# Autodesk Inventor assembly: x_motor
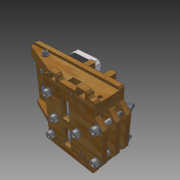
[picture p0: Inventor's stored thumbnail of the model, 180x180]
Saved by Autodesk Inventor 2014 (Build 180170000, 170)
## iProperties
Created: 2014-04-03
Part Number: x_motor
Document SubType Name: Assembly
Designer: buben
Author: buben
## Documents named in this file (23)
- C:\Users\buben\Documents\GitHub\bacon\inventor files\assemblies\x_motor.iam
- C:\Users\buben\Documents\GitHub\bacon\inventor files\printer parts\x_motor_back.ipt
- C:\Users\buben\Documents\GitHub\bacon\inventor files\printer parts\x_motor_cable_mount.ipt
- C:\Users\buben\Documents\GitHub\bacon\inventor files\printer parts\x_motor_cable_mount_brace.ipt
- C:\Users\buben\Documents\GitHub\bacon\inventor files\printer parts\x_motor_smooth_rod_spacer.ipt
- C:\Users\buben\Documents\GitHub\bacon\inventor files\printer parts\x_motor_wall_upper.ipt
- C:\Users\buben\Documents\GitHub\bacon\inventor files\printer parts\x_motor_wall_lower.ipt
- C:\Users\buben\Documents\GitHub\bacon\inventor files\printer parts\x_motor_upper_nut_stop.ipt
- C:\Users\buben\Documents\GitHub\bacon\inventor files\printer parts\motor_spacer.ipt
- C:\Users\buben\Documents\GitHub\bacon\inventor files\utils\washer_m4.ipt
- C:\Users\buben\Documents\Inventor\Content Center Files\R2014\en-US\ISO 4762(2)\ISO 4762 - M4 x 20ISO.ipt
- C:\Users\buben\Documents\Inventor\Content Center Files\R2014\en-US\ISO 7040\ISO 7040 - M4.ipt
- C:\Users\buben\Documents\GitHub\bacon\inventor files\printer parts\x_motor_middle.ipt
- C:\Users\buben\Documents\Inventor\Content Center Files\R2014\en-US\CSN EN 24032\ISO 4032 - M5CSN EN.ipt
- C:\Users\buben\Documents\GitHub\bacon\inventor files\3rd party components\linear_bearing_8\Imported Components\LU8MM\LU8MM.iam
- C:\Users\buben\Documents\GitHub\bacon\inventor files\printer parts\x_motor_top.ipt
- C:\Users\buben\Documents\GitHub\bacon\inventor files\printer parts\x_motor_lower_nut_stop.ipt
- C:\Users\buben\Documents\GitHub\bacon\inventor files\utils\washer_m5.ipt
- C:\Users\buben\Documents\Inventor\Content Center Files\R2014\en-US\ISO 7040\ISO 7040 - M5.ipt
- C:\Users\buben\Documents\Inventor\Content Center Files\R2014\en-US\ISO 4762(2)\ISO 4762 - M5 x 50ISO.ipt
- C:\Users\buben\Documents\GitHub\bacon\inventor files\utils\washer_m3.ipt
- C:\Users\buben\Documents\Inventor\Content Center Files\R2014\en-US\ISO 4762(2)\ISO 4762 - M3 x 20ISO.ipt
- C:\Users\buben\Documents\GitHub\bacon\inventor files\3rd party components\nema_17_stepper\Imported Components\NEMA 17 with T5 Pulley\NEMA 17 with T5 Pulley.iam
## Components (77 placed, 22 different names)
1. x_motor_back:1 — Mate:1, Mate:2, Mate:3, Mate:4, Mate:5, Mate:6, Mate:8, Mate:10, Mate:11, Mate:12, Mate:13, Mate:14, Mate:15, Mate:16, Mate:17, Mate:18, Mate:19, Mate:20, Mate:21, Mate:22, Mate:23, Mate:24, Mate:25, Tangent:1, Tangent:2, Mate:26, Mate:27, Mate:40, Mate:41, Mate:74, Mate:75, Mate:76, Mate:77, Mate:78, Mate:79, Mate:106, Mate:109, Mate:112, Mate:115
2. x_motor_cable_mount:1 — Mate:4, Mate:5, Mate:6, Mate:7, Mate:9, Mate:30, Mate:38, Mate:39
3. x_motor_cable_mount_brace:1 — Mate:7, Mate:8, Mate:9, Mate:42, Mate:44
4. x_motor_smooth_rod_spacer:1 — Mate:10, Mate:13, Mate:14
5. x_motor_smooth_rod_spacer:2 — Mate:11, Mate:12, Mate:15
6. x_motor_wall_upper:1 — Mate:16, Mate:17, Mate:18, Mate:32, Mate:50, Mate:54, Mate:55
7. x_motor_wall_lower:1 — Mate:19, Mate:20, Mate:21, Mate:51, Mate:52, Mate:56, Mate:57, Flush:1, Mate:63, Mate:64, Mate:67, Flush:2, Mate:125, Mate:126, Mate:127, Mate:128
8. x_motor_upper_nut_stop:1 — Mate:22, Mate:23, Mate:24, Mate:28, Mate:29, Mate:53
9. motor_spacer:1 — Mate:25, Tangent:1, Tangent:2, Mate:116, Mate:117, Mate:118, Mate:119, Mate:120, Mate:121, Mate:122
10. CSN 02 1702 B B 4,3:1 — Mate:28, Mate:29, Insert:1
11. CSN 02 1702 B B 4,3:2 — Mate:26, Mate:27, Insert:2
12. CSN 02 1702 B B 4,3:3 — Mate:32, Mate:33, Mate:34
13. CSN 02 1702 B B 4,3:4 — Mate:30, Mate:31, Mate:36
14. ISO 4762 M4 x 20:1 — Insert:2, Mate:31, Mate:37
15. ISO 4762 M4 x 20:2 — Insert:1, Mate:33, Mate:35
16. DIN EN ISO 7040 M4:1 — Mate:36, Mate:37
17. DIN EN ISO 7040 M4:2 — Mate:34, Mate:35
18. CSN 02 1702 B B 4,3:5 — Mate:44, Mate:45, Mate:48
19. CSN 02 1702 B B 4,3:6 — Mate:42, Mate:43, Mate:46
20. CSN 02 1702 B B 4,3:7 — Mate:38, Mate:39, Insert:4
21. CSN 02 1702 B B 4,3:8 — Mate:40, Mate:41, Insert:3
22. ISO 4762 M4 x 20:3 — Insert:4, Mate:43, Mate:47
23. ISO 4762 M4 x 20:4 — Insert:3, Mate:45, Mate:49
24. DIN EN ISO 7040 M4:3 — Mate:48, Mate:49
25. DIN EN ISO 7040 M4:4 — Mate:46, Mate:47
26. x_motor_middle:1 — Mate:50, Mate:51, Mate:52, Mate:58, Mate:59, Mate:60, Mate:62, Mate:66
27. CSN EN 24032 M5:1 — Mate:53, Mate:54, Mate:55
28. CSN EN 24032 M5:2 — Mate:56, Mate:57, Flush:1
29. LU8MM:1 [sub-assembly] — Mate:58, Mate:59, Mate:60, Mate:61
30. LU8MM:2 [sub-assembly] — Mate:61, Mate:62, Mate:65
31. x_motor_top:1 — Mate:63, Mate:64, Mate:65, Mate:68, Mate:69, Mate:70, Mate:71, Mate:72, Mate:73, Mate:80, Mate:81, Mate:82, Mate:83, Mate:84, Mate:85
32. x_motor_lower_nut_stop:1 — Mate:66, Mate:67, Flush:2, Mate:123, Mate:124
33. CSN 02 1702 B B 5,3:1 — Mate:72, Mate:83, Insert:7
34. CSN 02 1702 B B 5,3:2 — Mate:76, Mate:87, Mate:94
35. CSN 02 1702 B B 5,3:3 — Mate:77, Mate:91, Mate:102
36. CSN 02 1702 B B 5,3:4 — Mate:79, Mate:89, Mate:100
37. CSN 02 1702 B B 5,3:5 — Mate:78, Mate:90, Mate:98
38. CSN 02 1702 B B 5,3:6 — Mate:75, Mate:88, Mate:96
39. CSN 02 1702 B B 5,3:7 — Mate:74, Mate:86, Mate:92
40. CSN 02 1702 B B 5,3:8 — Mate:73, Mate:84, Insert:5
41. CSN 02 1702 B B 5,3:9 — Mate:71, Mate:85, Insert:9
42. CSN 02 1702 B B 5,3:10 — Mate:70, Mate:82, Insert:10
43. CSN 02 1702 B B 5,3:11 — Mate:69, Mate:81, Insert:8
44. CSN 02 1702 B B 5,3:12 — Mate:68, Mate:80, Insert:6
45. ISO 4762 M5 x 50:1 — Insert:10, Mate:86, Mate:93
46. ISO 4762 M5 x 50:4 — Insert:9, Mate:89, Mate:101
47. ISO 4762 M5 x 50:3 — Insert:8, Mate:88, Mate:97
48. ISO 4762 M5 x 50:5 — Insert:7, Mate:90, Mate:99
49. ISO 4762 M5 x 50:2 — Insert:6, Mate:87, Mate:95
50. ISO 4762 M5 x 50:6 — Insert:5, Mate:91, Mate:103
51. DIN EN ISO 7040 M5:1 — Mate:100, Mate:101
52. DIN EN ISO 7040 M5:2 — Mate:98, Mate:99
53. DIN EN ISO 7040 M5:3 — Mate:96, Mate:97
54. DIN EN ISO 7040 M5:4 — Mate:92, Mate:93
55. DIN EN ISO 7040 M5:5 — Mate:102, Mate:103
56. DIN EN ISO 7040 M5:6 — Mate:94, Mate:95
57. CSN 02 1702 B B 3,2:1 — Mate:110, Mate:111, Insert:13
58. CSN 02 1702 B B 3,2:2 — Mate:107, Mate:108, Insert:12
59. CSN 02 1702 B B 3,2:3 — Mate:110, Mate:111, Mate:112
60. CSN 02 1702 B B 3,2:4 — Mate:113, Mate:114, Insert:14
61. CSN 02 1702 B B 3,2:5 — Mate:113, Mate:114, Mate:115
62. CSN 02 1702 B B 3,2:6 — Mate:107, Mate:108, Mate:109
63. CSN 02 1702 B B 3,2:7 — Mate:104, Mate:105
64. CSN 02 1702 B B 3,2:8 — Mate:104, Mate:105, Mate:106, Insert:11
65. ISO 4762 M3 x 20:1 — Insert:14, Mate:122
66. ISO 4762 M3 x 20:2 — Insert:13, Mate:119
67. ISO 4762 M3 x 20:3 — Insert:12, Mate:120
68. ISO 4762 M3 x 20:4 — Insert:11, Mate:121
69. NEMA 17 with T5 Pulley:1 [sub-assembly] — Mate:116, Mate:117, Mate:118
70. CSN 02 1702 B B 4,3:9 — Mate:126, Mate:127, Insert:16
71. CSN 02 1702 B B 4,3:10 — Mate:125, Mate:128, Insert:15
72. CSN 02 1702 B B 4,3:11 — Mate:124, Mate:130, Mate:133
73. CSN 02 1702 B B 4,3:12 — Mate:123, Mate:129, Mate:131
74. ISO 4762 M4 x 20:5 — Insert:16, Mate:130, Mate:134
75. ISO 4762 M4 x 20:6 — Insert:15, Mate:129, Mate:132
76. DIN EN ISO 7040 M4:5 — Mate:133, Mate:134
77. DIN EN ISO 7040 M4:6 — Mate:131, Mate:132
## Relationships (154: Mate 134, Insert 16, Tangent 2, Flush 2)
- Mate:1: x_motor_back:1
- Mate:2: x_motor_back:1
- Mate:3: x_motor_back:1
- Mate:4: x_motor_back:1 ↔ x_motor_cable_mount:1
- Mate:5: x_motor_back:1 ↔ x_motor_cable_mount:1
- Mate:6: x_motor_back:1 ↔ x_motor_cable_mount:1
- Mate:7: x_motor_cable_mount:1 ↔ x_motor_cable_mount_brace:1
- Mate:8: x_motor_back:1 ↔ x_motor_cable_mount_brace:1
- Mate:9: x_motor_cable_mount:1 ↔ x_motor_cable_mount_brace:1
- Mate:10: x_motor_back:1 ↔ x_motor_smooth_rod_spacer:1
- Mate:11: x_motor_back:1 ↔ x_motor_smooth_rod_spacer:2
- Mate:12: x_motor_back:1 ↔ x_motor_smooth_rod_spacer:2
- Mate:13: x_motor_back:1 ↔ x_motor_smooth_rod_spacer:1
- Mate:14: x_motor_back:1 ↔ x_motor_smooth_rod_spacer:1
- Mate:15: x_motor_back:1 ↔ x_motor_smooth_rod_spacer:2
- Mate:16: x_motor_back:1 ↔ x_motor_wall_upper:1
- Mate:17: x_motor_back:1 ↔ x_motor_wall_upper:1
- Mate:18: x_motor_back:1 ↔ x_motor_wall_upper:1
- Mate:19: x_motor_back:1 ↔ x_motor_wall_lower:1
- Mate:20: x_motor_back:1 ↔ x_motor_wall_lower:1
- Mate:21: x_motor_back:1 ↔ x_motor_wall_lower:1
- Mate:22: x_motor_back:1 ↔ x_motor_upper_nut_stop:1
- Mate:23: x_motor_back:1 ↔ x_motor_upper_nut_stop:1
- Mate:24: x_motor_back:1 ↔ x_motor_upper_nut_stop:1
- Mate:25: x_motor_back:1 ↔ motor_spacer:1
- Tangent:1: x_motor_back:1 ↔ motor_spacer:1
- Tangent:2: x_motor_back:1 ↔ motor_spacer:1
- Mate:26: x_motor_back:1 ↔ CSN 02 1702 B B 4,3:2
- Mate:27: x_motor_back:1 ↔ CSN 02 1702 B B 4,3:2
- Mate:28: x_motor_upper_nut_stop:1 ↔ CSN 02 1702 B B 4,3:1
- Mate:29: x_motor_upper_nut_stop:1 ↔ CSN 02 1702 B B 4,3:1
- Insert:1: CSN 02 1702 B B 4,3:1 ↔ ISO 4762 M4 x 20:2
- Insert:2: CSN 02 1702 B B 4,3:2 ↔ ISO 4762 M4 x 20:1
- Mate:30: x_motor_cable_mount:1 ↔ CSN 02 1702 B B 4,3:4
- Mate:31: CSN 02 1702 B B 4,3:4 ↔ ISO 4762 M4 x 20:1
- Mate:32: x_motor_wall_upper:1 ↔ CSN 02 1702 B B 4,3:3
- Mate:33: CSN 02 1702 B B 4,3:3 ↔ ISO 4762 M4 x 20:2
- Mate:34: CSN 02 1702 B B 4,3:3 ↔ DIN EN ISO 7040 M4:2
- Mate:35: ISO 4762 M4 x 20:2 ↔ DIN EN ISO 7040 M4:2
- Mate:36: CSN 02 1702 B B 4,3:4 ↔ DIN EN ISO 7040 M4:1
- Mate:37: ISO 4762 M4 x 20:1 ↔ DIN EN ISO 7040 M4:1
- Mate:38: x_motor_cable_mount:1 ↔ CSN 02 1702 B B 4,3:7
- Mate:39: x_motor_cable_mount:1 ↔ CSN 02 1702 B B 4,3:7
- Mate:40: x_motor_back:1 ↔ CSN 02 1702 B B 4,3:8
- Mate:41: x_motor_back:1 ↔ CSN 02 1702 B B 4,3:8
- Insert:3: CSN 02 1702 B B 4,3:8 ↔ ISO 4762 M4 x 20:4
- Insert:4: CSN 02 1702 B B 4,3:7 ↔ ISO 4762 M4 x 20:3
- Mate:42: x_motor_cable_mount_brace:1 ↔ CSN 02 1702 B B 4,3:6
- Mate:43: CSN 02 1702 B B 4,3:6 ↔ ISO 4762 M4 x 20:3
- Mate:44: x_motor_cable_mount_brace:1 ↔ CSN 02 1702 B B 4,3:5
- Mate:45: CSN 02 1702 B B 4,3:5 ↔ ISO 4762 M4 x 20:4
- Mate:46: CSN 02 1702 B B 4,3:6 ↔ DIN EN ISO 7040 M4:4
- Mate:47: ISO 4762 M4 x 20:3 ↔ DIN EN ISO 7040 M4:4
- Mate:48: CSN 02 1702 B B 4,3:5 ↔ DIN EN ISO 7040 M4:3
- Mate:49: ISO 4762 M4 x 20:4 ↔ DIN EN ISO 7040 M4:3
- Mate:50: x_motor_wall_upper:1 ↔ x_motor_middle:1
- Mate:51: x_motor_wall_lower:1 ↔ x_motor_middle:1
- Mate:52: x_motor_wall_lower:1 ↔ x_motor_middle:1
- Mate:53: x_motor_upper_nut_stop:1 ↔ CSN EN 24032 M5:1
- Mate:54: x_motor_wall_upper:1 ↔ CSN EN 24032 M5:1
- Mate:55: x_motor_wall_upper:1 ↔ CSN EN 24032 M5:1
- Mate:56: x_motor_wall_lower:1 ↔ CSN EN 24032 M5:2
- Mate:57: x_motor_wall_lower:1 ↔ CSN EN 24032 M5:2
- Flush:1: x_motor_wall_lower:1 ↔ CSN EN 24032 M5:2
- Mate:58 (7.5 mm): x_motor_middle:1 ↔ LU8MM:1
- Mate:59 (7.5 mm): x_motor_middle:1 ↔ LU8MM:1
- Mate:60 (0.5 mm): x_motor_middle:1 ↔ LU8MM:1
- Mate:61: LU8MM:1 ↔ LU8MM:2
- Mate:62 (0.5 mm): x_motor_middle:1 ↔ LU8MM:2
- Mate:63: x_motor_wall_lower:1 ↔ x_motor_top:1
- Mate:64: x_motor_wall_lower:1 ↔ x_motor_top:1
- Mate:65 (7.5 mm): LU8MM:2 ↔ x_motor_top:1
- Mate:66: x_motor_middle:1 ↔ x_motor_lower_nut_stop:1
- Mate:67: x_motor_wall_lower:1 ↔ x_motor_lower_nut_stop:1
- Flush:2: x_motor_wall_lower:1 ↔ x_motor_lower_nut_stop:1
- Mate:68: x_motor_top:1 ↔ CSN 02 1702 B B 5,3:12
- Mate:69: x_motor_top:1 ↔ CSN 02 1702 B B 5,3:11
- Mate:70: x_motor_top:1 ↔ CSN 02 1702 B B 5,3:10
- Mate:71: x_motor_top:1 ↔ CSN 02 1702 B B 5,3:9
- Mate:72: x_motor_top:1 ↔ CSN 02 1702 B B 5,3:1
- Mate:73: x_motor_top:1 ↔ CSN 02 1702 B B 5,3:8
- Mate:74: x_motor_back:1 ↔ CSN 02 1702 B B 5,3:7
- Mate:75: x_motor_back:1 ↔ CSN 02 1702 B B 5,3:6
- Mate:76: x_motor_back:1 ↔ CSN 02 1702 B B 5,3:2
- Mate:77: x_motor_back:1 ↔ CSN 02 1702 B B 5,3:3
- Mate:78: x_motor_back:1 ↔ CSN 02 1702 B B 5,3:5
- Mate:79: x_motor_back:1 ↔ CSN 02 1702 B B 5,3:4
- Mate:80: x_motor_top:1 ↔ CSN 02 1702 B B 5,3:12
- Mate:81: x_motor_top:1 ↔ CSN 02 1702 B B 5,3:11
- Mate:82: x_motor_top:1 ↔ CSN 02 1702 B B 5,3:10
- Mate:83: x_motor_top:1 ↔ CSN 02 1702 B B 5,3:1
- Mate:84: x_motor_top:1 ↔ CSN 02 1702 B B 5,3:8
- Mate:85: x_motor_top:1 ↔ CSN 02 1702 B B 5,3:9
- Insert:5: CSN 02 1702 B B 5,3:8 ↔ ISO 4762 M5 x 50:6
- Insert:6: CSN 02 1702 B B 5,3:12 ↔ ISO 4762 M5 x 50:2
- Insert:7: CSN 02 1702 B B 5,3:1 ↔ ISO 4762 M5 x 50:5
- Insert:8: CSN 02 1702 B B 5,3:11 ↔ ISO 4762 M5 x 50:3
- Insert:9: CSN 02 1702 B B 5,3:9 ↔ ISO 4762 M5 x 50:4
- Insert:10: CSN 02 1702 B B 5,3:10 ↔ ISO 4762 M5 x 50:1
- Mate:86: CSN 02 1702 B B 5,3:7 ↔ ISO 4762 M5 x 50:1
- Mate:87: CSN 02 1702 B B 5,3:2 ↔ ISO 4762 M5 x 50:2
- Mate:88: CSN 02 1702 B B 5,3:6 ↔ ISO 4762 M5 x 50:3
- Mate:89: CSN 02 1702 B B 5,3:4 ↔ ISO 4762 M5 x 50:4
- Mate:90: CSN 02 1702 B B 5,3:5 ↔ ISO 4762 M5 x 50:5
- Mate:91: CSN 02 1702 B B 5,3:3 ↔ ISO 4762 M5 x 50:6
- Mate:92: CSN 02 1702 B B 5,3:7 ↔ DIN EN ISO 7040 M5:4
- Mate:93: ISO 4762 M5 x 50:1 ↔ DIN EN ISO 7040 M5:4
- Mate:94: CSN 02 1702 B B 5,3:2 ↔ DIN EN ISO 7040 M5:6
- Mate:95: ISO 4762 M5 x 50:2 ↔ DIN EN ISO 7040 M5:6
- Mate:96: CSN 02 1702 B B 5,3:6 ↔ DIN EN ISO 7040 M5:3
- Mate:97: ISO 4762 M5 x 50:3 ↔ DIN EN ISO 7040 M5:3
- Mate:98: CSN 02 1702 B B 5,3:5 ↔ DIN EN ISO 7040 M5:2
- Mate:99: ISO 4762 M5 x 50:5 ↔ DIN EN ISO 7040 M5:2
- Mate:100: CSN 02 1702 B B 5,3:4 ↔ DIN EN ISO 7040 M5:1
- Mate:101: ISO 4762 M5 x 50:4 ↔ DIN EN ISO 7040 M5:1
- Mate:102: CSN 02 1702 B B 5,3:3 ↔ DIN EN ISO 7040 M5:5
- Mate:103: ISO 4762 M5 x 50:6 ↔ DIN EN ISO 7040 M5:5
- Mate:104: CSN 02 1702 B B 3,2:7 ↔ CSN 02 1702 B B 3,2:8
- Mate:105: CSN 02 1702 B B 3,2:7 ↔ CSN 02 1702 B B 3,2:8
- Mate:106: x_motor_back:1 ↔ CSN 02 1702 B B 3,2:8
- Mate:107: CSN 02 1702 B B 3,2:2 ↔ CSN 02 1702 B B 3,2:6
- Mate:108: CSN 02 1702 B B 3,2:2 ↔ CSN 02 1702 B B 3,2:6
- Mate:109: x_motor_back:1 ↔ CSN 02 1702 B B 3,2:6
- Mate:110: CSN 02 1702 B B 3,2:1 ↔ CSN 02 1702 B B 3,2:3
- Mate:111: CSN 02 1702 B B 3,2:1 ↔ CSN 02 1702 B B 3,2:3
- Mate:112: x_motor_back:1 ↔ CSN 02 1702 B B 3,2:3
- Mate:113: CSN 02 1702 B B 3,2:4 ↔ CSN 02 1702 B B 3,2:5
- Mate:114: CSN 02 1702 B B 3,2:4 ↔ CSN 02 1702 B B 3,2:5
- Mate:115: x_motor_back:1 ↔ CSN 02 1702 B B 3,2:5
- Insert:11: CSN 02 1702 B B 3,2:8 ↔ ISO 4762 M3 x 20:4
- Insert:12: CSN 02 1702 B B 3,2:2 ↔ ISO 4762 M3 x 20:3
- Insert:13: CSN 02 1702 B B 3,2:1 ↔ ISO 4762 M3 x 20:2
- Insert:14: CSN 02 1702 B B 3,2:4 ↔ ISO 4762 M3 x 20:1
- Mate:116: motor_spacer:1 ↔ NEMA 17 with T5 Pulley:1
- Mate:117: motor_spacer:1 ↔ NEMA 17 with T5 Pulley:1
- Mate:118: motor_spacer:1 ↔ NEMA 17 with T5 Pulley:1
- Mate:119: motor_spacer:1 ↔ ISO 4762 M3 x 20:2
- Mate:120: motor_spacer:1 ↔ ISO 4762 M3 x 20:3
- Mate:121: motor_spacer:1 ↔ ISO 4762 M3 x 20:4
- Mate:122: motor_spacer:1 ↔ ISO 4762 M3 x 20:1
- Mate:123: x_motor_lower_nut_stop:1 ↔ CSN 02 1702 B B 4,3:12
- Mate:124: x_motor_lower_nut_stop:1 ↔ CSN 02 1702 B B 4,3:11
- Mate:125: x_motor_wall_lower:1 ↔ CSN 02 1702 B B 4,3:10
- Mate:126: x_motor_wall_lower:1 ↔ CSN 02 1702 B B 4,3:9
- Mate:127: x_motor_wall_lower:1 ↔ CSN 02 1702 B B 4,3:9
- Mate:128: x_motor_wall_lower:1 ↔ CSN 02 1702 B B 4,3:10
- Insert:15: CSN 02 1702 B B 4,3:10 ↔ ISO 4762 M4 x 20:6
- Insert:16: CSN 02 1702 B B 4,3:9 ↔ ISO 4762 M4 x 20:5
- Mate:129: CSN 02 1702 B B 4,3:12 ↔ ISO 4762 M4 x 20:6
- Mate:130: CSN 02 1702 B B 4,3:11 ↔ ISO 4762 M4 x 20:5
- Mate:131: CSN 02 1702 B B 4,3:12 ↔ DIN EN ISO 7040 M4:6
- Mate:132: ISO 4762 M4 x 20:6 ↔ DIN EN ISO 7040 M4:6
- Mate:133: CSN 02 1702 B B 4,3:11 ↔ DIN EN ISO 7040 M4:5
- Mate:134: ISO 4762 M4 x 20:5 ↔ DIN EN ISO 7040 M4:5
